# Autodesk Inventor assembly: Thigh
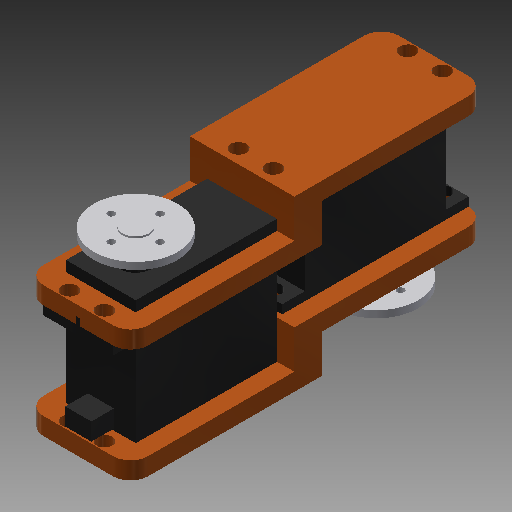
[picture p0: Inventor's stored thumbnail of the model, 512x512]
Saved by Autodesk Inventor 2017 (Build 210142000, 142)
## iProperties
Created: 2017-01-25
Part Number: Thigh
Document SubType Name: Assembly
Designer: Alexander Miller
Author: Alexander Miller
## Documents named in this file (3)
- D:\Daten\Documents\Git\Hexapod\3DParts\HexPi_v2\Thigh.iam
- D:\Daten\Documents\Git\Hexapod\3DParts\HexPi_v2\Serov_with_arm.iam
- D:\Daten\Documents\Git\Hexapod\3DParts\HexPi_v2\Femur_c.ipt
## Components (4 placed, 2 different names)
1. Serov_with_arm:1 [sub-assembly] — Rigid:2, Rigid:3
2. Serov_with_arm:2 [sub-assembly] — Rigid:1
3. Femur_c:1 — Rigid:1, Rigid:3
4. Femur_c:2 — Rigid:2
## Relationships (3: WeldJoint 3)
- Rigid:1 [WeldJoint]: Serov_with_arm:2 ↔ Femur_c:1
- Rigid:2 [WeldJoint]: Serov_with_arm:1 ↔ Femur_c:2
- Rigid:3 [WeldJoint]: Serov_with_arm:1 ↔ Femur_c:1
